# Autodesk Inventor assembly: marco
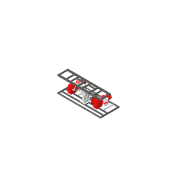
[picture p0: Inventor's stored thumbnail of the model, 180x180]
Saved by Autodesk Inventor 2021 (Build 250183000, 183)
## iProperties
Created: 2021-04-11
Part Number: marco
Document SubType Name: Assembly
Designer: equip
Mass: 593990 g
Surface Area: 185574 cm^2
Volume: 307928 cm^3
Density: 1.92899 g/cm^3
_SolveAssemblyDoc: Frame Generator Solve Assembly
_Version: 25.0.0
Author: equip
## Documents named in this file (19)
- C:\Users\Santiago Suárez\Documents\GitHub\Dis.-Mecatronico-E6\inventor proyecto\EnsambleGeneral.iam
- C:\Users\Santiago Suárez\Documents\GitHub\Dis.-Mecatronico-E6\inventor proyecto\Silla del marco.ipt
- C:\Users\Santiago Suárez\Documents\GitHub\Dis.-Mecatronico-E6\inventor proyecto\marco inferior.ipt
- C:\Users\Santiago Suárez\Documents\GitHub\Dis.-Mecatronico-E6\inventor proyecto\marco\Frame\Marco Inferior.iam
- C:\Users\Santiago Suárez\Documents\GitHub\Dis.-Mecatronico-E6\inventor proyecto\MarcoSuperior.iam
- C:\Users\Santiago Suárez\Documents\GitHub\Dis.-Mecatronico-E6\inventor proyecto\PlacaInferior.ipt
- C:\Users\Santiago Suárez\Documents\GitHub\Dis.-Mecatronico-E6\inventor proyecto\DSV Sitting.iam
- C:\Users\Santiago Suárez\Documents\GitHub\Dis.-Mecatronico-E6\inventor proyecto\PARTserver0202108060004321756159710e898ce\AIS2021\574118 ESBF-BS-100-100-20P---(0).iam
- C:\Users\Santiago Suárez\Documents\GitHub\Dis.-Mecatronico-E6\inventor proyecto\Motores y reductores\Sistema movimiento derecho.iam
- C:\Users\Santiago Suárez\Documents\GitHub\Dis.-Mecatronico-E6\inventor proyecto\Motores y reductores\Sistema movimiento izquierdo.iam
- C:\Users\Santiago Suárez\Documents\GitHub\Dis.-Mecatronico-E6\inventor proyecto\UnionMarco.ipt
- C:\Users\Santiago Suárez\Documents\GitHub\Dis.-Mecatronico-E6\inventor proyecto\Eje.ipt
- C:\Users\Santiago Suárez\Documents\GitHub\Dis.-Mecatronico-E6\inventor proyecto\BaseMotor.ipt
- C:\Users\Santiago Suárez\Documents\GitHub\Dis.-Mecatronico-E6\inventor proyecto\marco\AIP\FEA\dn6km6b1c.fins
- C:\Users\Santiago Suárez\Documents\GitHub\Dis.-Mecatronico-E6\inventor proyecto\marco\AIP\FEA\dn6km6b1c.fsat
- C:\Users\Santiago Suárez\Documents\GitHub\Dis.-Mecatronico-E6\inventor proyecto\marco\AIP\FEA\dn6km6b1c.ftes
- C:\Users\Santiago Suárez\Documents\GitHub\Dis.-Mecatronico-E6\inventor proyecto\marco\AIP\FEA\dn6km6b1c.fwiz
- C:\Users\Santiago Suárez\Documents\GitHub\Dis.-Mecatronico-E6\inventor proyecto\marco\AIP\FEA\dn6km6b5s.fmsh
- C:\Users\Santiago Suárez\Documents\GitHub\Dis.-Mecatronico-E6\inventor proyecto\marco\AIP\FEA\dn6km6b5t.fres
## Components (21 placed, 12 different names)
1. marco inferior:1
2. Marco Inferior:1 [sub-assembly] — Mate:39, Mate:40, Flush:1, Mate:41, Mate:42, Mate:46, Mate:49, Mate:50, Mate:57, Flush:46
3. MarcoSuperior:1 [sub-assembly] — Rigid:3, Mate:35, Mate:36, Mate:37, Mate:47, Mate:48, Mate:51, Mate:52, Mate:53, Mate:54
4. PlacaInferior:1 — Mate:38, Flush:45, Mate:46, Mate:49, Mate:50, Flush:2
5. DSV Sitting:1 [sub-assembly] — Rigid:17
6. DSV Sitting:2 [sub-assembly] — Rigid:20
7. DSV Sitting:3 [sub-assembly] — Rigid:19
8. DSV Sitting:4 [sub-assembly] — Rigid:18
9. 574118 ESBF-BS-100-100-20P---(0):1 [sub-assembly] — Mate:38, Flush:45, Flush:2, Rigid:3
10. Sistema movimiento derecho:1 [sub-assembly] — Mate:40, Flush:1, Mate:41, Mate:57, Rigid:21, Insert:2
11. Sistema movimiento izquierdo:1 [sub-assembly] — Mate:39, Mate:42, Flush:46, Rigid:22, Insert:1
12. UnionMarco:1 — Mate:47, Mate:48, Mate:51, Mate:55, Flush:3, Insert:1
13. UnionMarco:2 — Mate:52, Mate:53, Mate:54, Mate:56, Flush:4
14. Eje:1 — Mate:55, Flush:3
15. Eje:2 — Mate:56, Flush:4, Insert:2
16. BaseMotor:1 — Rigid:22
17. BaseMotor:2 — Rigid:21
18. Silla del marco:1 — Rigid:17, Mate:35, Mate:36, Mate:37
19. Silla del marco:2 — Rigid:18
20. Silla del marco:3 — Rigid:19
21. Silla del marco:4 — Rigid:20
## Component patterns: (4 elements, first: Silla del marco:1)
## Relationships (35: Mate 20, WeldJoint 7, Flush 6, Insert 2)
- Rigid:3 [WeldJoint]: MarcoSuperior:1 ↔ 574118 ESBF-BS-100-100-20P---(0):1
- Rigid:17 [WeldJoint] (-40 mm): DSV Sitting:1 ↔ Silla del marco:1
- Rigid:18 [WeldJoint] (-40 mm): DSV Sitting:4 ↔ Silla del marco:2
- Rigid:19 [WeldJoint] (-40 mm): DSV Sitting:3 ↔ Silla del marco:3
- Rigid:20 [WeldJoint] (-40 mm): DSV Sitting:2 ↔ Silla del marco:4
- Mate:35: MarcoSuperior:1 ↔ Silla del marco:1
- Mate:36: MarcoSuperior:1 ↔ Silla del marco:1
- Mate:37: MarcoSuperior:1 ↔ Silla del marco:1
- Mate:38: PlacaInferior:1 ↔ 574118 ESBF-BS-100-100-20P---(0):1
- Mate:39 (100 mm): Marco Inferior:1 ↔ Sistema movimiento izquierdo:1
- Mate:40: Marco Inferior:1 ↔ Sistema movimiento derecho:1
- Flush:1: Marco Inferior:1 ↔ Sistema movimiento derecho:1
- Mate:41 (338 mm): Marco Inferior:1 ↔ Sistema movimiento derecho:1
- Mate:42 (338 mm): Marco Inferior:1 ↔ Sistema movimiento izquierdo:1
- Flush:45 (65.3 mm): PlacaInferior:1 ↔ 574118 ESBF-BS-100-100-20P---(0):1
- Mate:46: Marco Inferior:1 ↔ PlacaInferior:1
- Mate:47: MarcoSuperior:1 ↔ UnionMarco:1
- Mate:48: MarcoSuperior:1 ↔ UnionMarco:1
- Mate:49: Marco Inferior:1 ↔ PlacaInferior:1
- Mate:50: Marco Inferior:1 ↔ PlacaInferior:1
- Flush:2 (44 mm): PlacaInferior:1 ↔ 574118 ESBF-BS-100-100-20P---(0):1
- Mate:51 (252 mm): MarcoSuperior:1 ↔ UnionMarco:1
- Mate:52: MarcoSuperior:1 ↔ UnionMarco:2
- Mate:53: MarcoSuperior:1 ↔ UnionMarco:2
- Mate:54 (252 mm): MarcoSuperior:1 ↔ UnionMarco:2
- Mate:55: UnionMarco:1 ↔ Eje:1
- Flush:3 (-18.5 mm): UnionMarco:1 ↔ Eje:1
- Mate:56: UnionMarco:2 ↔ Eje:2
- Flush:4 (-18.5 mm): UnionMarco:2 ↔ Eje:2
- Mate:57 (100 mm): Marco Inferior:1 ↔ Sistema movimiento derecho:1
- Flush:46: Marco Inferior:1 ↔ Sistema movimiento izquierdo:1
- Rigid:21 [WeldJoint]: Sistema movimiento derecho:1 ↔ BaseMotor:2
- Rigid:22 [WeldJoint]: Sistema movimiento izquierdo:1 ↔ BaseMotor:1
- Insert:1 (1.5 mm): Sistema movimiento izquierdo:1 ↔ UnionMarco:1
- Insert:2 (25 mm): Sistema movimiento derecho:1 ↔ Eje:2
## Named parameters: sa_0 = 69000, sa_1 = 69000, sa_2 = 69000, sa_3 = 69000, sa_4 = 69000, sa_5 = 69000, sa_6 = 69000, sa_7 = 69000
note: some values were not read from the file. Shown as the stored number, unit unknown: "sa_0", "sa_1", "sa_2", "sa_3", "sa_4", "sa_5", "sa_6", "sa_7".
